# Autodesk Inventor assembly: check_mid_assembly
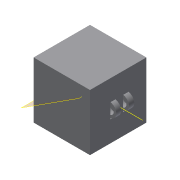
[picture p0: Inventor's stored thumbnail of the model, 180x180]
Saved by Autodesk Inventor 2017 (Build 210142000, 142)
## iProperties
Created: 2018-07-13
Part Number: check_mid_assembly
Document SubType Name: Assembly
Designer: Nic
Author: Nic
## Documents named in this file (4)
- C:\Users\Nic\Documents\Antenna\check_mid_assembly.iam
- C:\Users\Nic\Documents\Antenna\mould_casing_base_v3.ipt
- C:\Users\Nic\Documents\Antenna\middle_segment_v3.ipt
- C:\Users\Nic\Documents\Antenna\mould_casing_top_v3.ipt
## Components (3 placed, 3 different names)
1. mould_casing_base_v3:1 — Mate:1, Angle:1, Mate:2, Mate:3, Mate:4, Flush:1, Flush:2
2. middle_segment_v3:1 — Mate:1, Angle:1, Mate:2, Mate:3
3. mould_casing_top_v3:1 — Mate:4, Flush:1, Flush:2
## Relationships (7: Mate 4, Flush 2, Angle 1)
- Mate:1 (0.2 mm): mould_casing_base_v3:1 ↔ middle_segment_v3:1
- Angle:1 (0 deg): mould_casing_base_v3:1 ↔ middle_segment_v3:1
- Mate:2 (0.1 mm): mould_casing_base_v3:1 ↔ middle_segment_v3:1
- Mate:3 (0.2 mm): mould_casing_base_v3:1 ↔ middle_segment_v3:1
- Mate:4: mould_casing_base_v3:1 ↔ mould_casing_top_v3:1
- Flush:1: mould_casing_base_v3:1 ↔ mould_casing_top_v3:1
- Flush:2: mould_casing_base_v3:1 ↔ mould_casing_top_v3:1
